# Autodesk Inventor assembly: GP1-100
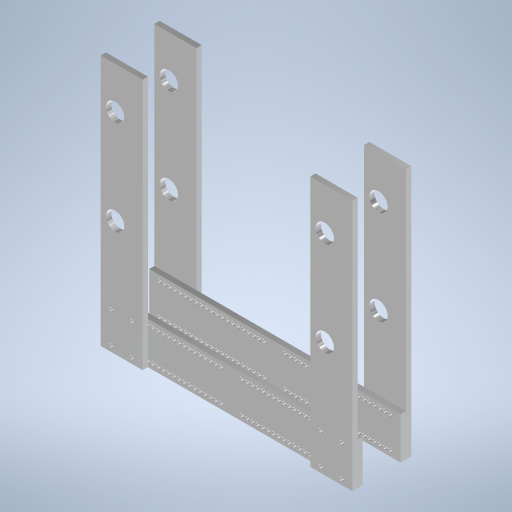
[picture p0: Inventor's stored thumbnail of the model, 512x512]
Saved by Autodesk Inventor 2023.4 (Build 274418000, 418)
## iProperties
Created: 2025-01-05
Part Number: GP1-100
Document SubType Name: Assembly
Designer: mavericks
Author: mavericks
## Documents named in this file (3)
- C:\Users\mavericks\Desktop\2025-ReefScape---CAD\Gripper\GP1-100.iam
- C:\Users\mavericks\Desktop\2025-ReefScape---CAD\Gripper\Gp1-001.ipt
- C:\Users\mavericks\Desktop\2025-ReefScape---CAD\Gripper\GP1-002.ipt
## Components (6 placed, 2 different names)
1. GP1-002:1 — Insert:5, Insert:6
2. GP1-002:2 — Insert:3, Insert:4
3. GP1-002:3 — Insert:1, Insert:2
4. GP1-002:4 — Insert:7, Insert:8
5. Gp1-001:2 — Insert:1, Insert:2, Insert:3, Insert:4, Flush:1, Flush:2
6. Gp1-001:3 — Insert:5, Insert:6, Insert:7, Insert:8, Flush:1, Flush:2
## Relationships (10: Insert 8, Flush 2)
- Insert:1: GP1-002:3 ↔ Gp1-001:2
- Insert:2: GP1-002:3 ↔ Gp1-001:2
- Insert:3: GP1-002:2 ↔ Gp1-001:2
- Insert:4: GP1-002:2 ↔ Gp1-001:2
- Insert:5: GP1-002:1 ↔ Gp1-001:3
- Insert:6: GP1-002:1 ↔ Gp1-001:3
- Insert:7: GP1-002:4 ↔ Gp1-001:3
- Insert:8: GP1-002:4 ↔ Gp1-001:3
- Flush:1: Gp1-001:2 ↔ Gp1-001:3
- Flush:2: Gp1-001:2 ↔ Gp1-001:3
